# Autodesk Inventor assembly: actuator assem
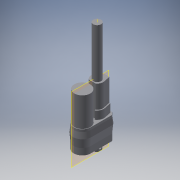
[picture p0: Inventor's stored thumbnail of the model, 180x180]
Saved by Autodesk Inventor 2018 (Build 220112000, 112)
## iProperties
Created: 2020-04-10
Part Number: actuator assem
Document SubType Name: Assembly
Designer: Jesse R-B
Author: Jesse R-B
## Documents named in this file (4)
- C:\Users\Jesse R-B\Documents\Inventor\400\V2\V3\actuator assem.iam
- C:\Users\Jesse R-B\Documents\Inventor\400\HDA-BASE.ipt
- C:\Users\Jesse R-B\Documents\Inventor\400\V2\V3\JlinearActuator1.ipt
- C:\Users\Jesse R-B\Documents\Inventor\400\V2\V3\acutatedpole.ipt
## Components (3 placed, 3 different names)
1. HDA-BASE:1 — Mate:1, Mate:2, Mate:3
2. JlinearActuator1:1 — Mate:1, Mate:2, Mate:3, Mate:4
3. acutatedpole:1 — Mate:4, Mate:5, Mate:6
## Relationships (6: Mate 6)
- Mate:1: HDA-BASE:1 ↔ JlinearActuator1:1
- Mate:2: HDA-BASE:1 ↔ JlinearActuator1:1
- Mate:3: HDA-BASE:1 ↔ JlinearActuator1:1
- Mate:4: JlinearActuator1:1 ↔ acutatedpole:1
- Mate:5: acutatedpole:1
- Mate:6: acutatedpole:1
